# Autodesk Inventor assembly: HeadUnit
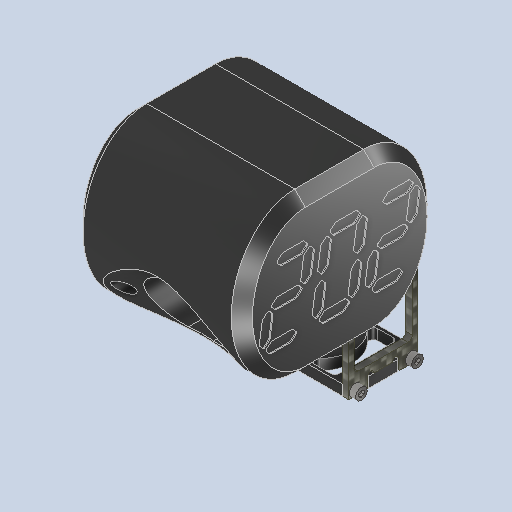
[picture p0: Inventor's stored thumbnail of the model, 512x512]
Saved by Autodesk Inventor 2024.2 (Build 282272000, 272)
## iProperties
Created: 2024-01-19
Part Number: HeadUnit
Document SubType Name: Assembly
Designer: Masato Kubotera
Mass: 257.797 g
Surface Area: 969.022 cm^2
Volume: 207.363 cm^3
Density: 1.24322 g/cm^3
Author: Masato Kubotera
## Documents named in this file (17)
- C:\Users\masato\OneDrive - Chiba Institute of Technology\CIT Brains\RoboCup2024\Mechanic\SUSTAINA-OP2-DEV - 作業\NativeFiles\Boby\Head\HeadUnit.iam
- C:\Users\masato\OneDrive - Chiba Institute of Technology\CIT Brains\RoboCup2024\Mechanic\SUSTAINA-OP2-DEV - 作業\NativeFiles\Boby\COTS\Screws\CapScrew\UC-0308.ipt
- C:\Users\masato\OneDrive - Chiba Institute of Technology\CIT Brains\RoboCup2024\Mechanic\SUSTAINA-OP2-DEV - 作業\NativeFiles\Boby\Head\HeadCameraMountFrame.ipt
- C:\Users\masato\OneDrive - Chiba Institute of Technology\CIT Brains\RoboCup2024\Mechanic\SUSTAINA-OP2-DEV - 作業\NativeFiles\Boby\Head\HeadHornFrame.ipt
- C:\Users\masato\OneDrive - Chiba Institute of Technology\CIT Brains\RoboCup2024\Mechanic\SUSTAINA-OP2-DEV - 作業\NativeFiles\Boby\Head\HeadSideFrame.ipt
- C:\Users\masato\OneDrive - Chiba Institute of Technology\CIT Brains\RoboCup2024\Mechanic\SUSTAINA-OP2-DEV - 作業\NativeFiles\Boby\COTS\Spacers\C-2006-4.ipt
- C:\Users\masato\OneDrive - Chiba Institute of Technology\CIT Brains\RoboCup2024\Mechanic\SUSTAINA-OP2-DEV - 作業\NativeFiles\Boby\Head\HeadSpeakerMountFrame.ipt
- C:\Users\masato\OneDrive - Chiba Institute of Technology\CIT Brains\RoboCup2024\Mechanic\SUSTAINA-OP2-DEV - 作業\NativeFiles\Boby\COTS\ElectronicComponents\CMS-402811-28SP.ipt
- C:\Users\masato\OneDrive - Chiba Institute of Technology\CIT Brains\RoboCup2024\Mechanic\SUSTAINA-OP2-DEV - 作業\NativeFiles\Boby\Head\HeadCircuitMountFrame.ipt
- C:\Users\masato\OneDrive - Chiba Institute of Technology\CIT Brains\RoboCup2024\Mechanic\SUSTAINA-OP2-DEV - 作業\NativeFiles\Boby\COTS\Screws\CapScrew\UC-0206.ipt
- C:\Users\masato\OneDrive - Chiba Institute of Technology\CIT Brains\RoboCup2024\Mechanic\SUSTAINA-OP2-DEV - 作業\NativeFiles\Boby\Head\HeadCover.ipt
- C:\Users\masato\OneDrive - Chiba Institute of Technology\CIT Brains\RoboCup2024\Mechanic\SUSTAINA-OP2-DEV - 作業\NativeFiles\Boby\COTS\ElectronicComponents\Cameras\e-CAM50_CUONX.ipt
- C:\Users\masato\OneDrive - Chiba Institute of Technology\CIT Brains\RoboCup2024\Mechanic\SUSTAINA-OP2-DEV - 作業\NativeFiles\Boby\COTS\Spacers\C-2002.5-4.ipt
- C:\Users\masato\OneDrive - Chiba Institute of Technology\CIT Brains\RoboCup2024\Mechanic\SUSTAINA-OP2-DEV - 作業\NativeFiles\Boby\COTS\Screws\CapScrew\FC-0215EB.ipt
- C:\Users\masato\OneDrive - Chiba Institute of Technology\CIT Brains\RoboCup2024\Mechanic\SUSTAINA-OP2-DEV - 作業\NativeFiles\Boby\CustomPCBs\SUSTAINA-SCI-TO-HDMI-BOARD.ipt
- C:\Users\masato\OneDrive - Chiba Institute of Technology\CIT Brains\RoboCup2024\Mechanic\SUSTAINA-OP2-DEV - 作業\NativeFiles\Boby\COTS\CIL926-F2.4-M12A650.ipt
- C:\Users\masato\OneDrive - Chiba Institute of Technology\CIT Brains\RoboCup2024\Mechanic\SUSTAINA-OP2-DEV - 作業\NativeFiles\Boby\COTS\Screws\CapScrew\UC-0310.ipt
## Components (50 placed, 16 different names)
1. HeadSpeakerMountFrame:1 — Insert:58, Insert:59, Insert:60, Insert:61, Insert:66, Insert:67, Insert:68, Insert:69
2. HeadCircuitMountFrame:1 — Insert:74, Insert:75, Insert:76, Insert:77, Insert:94, Insert:95
3. HeadCameraMountFrame:1 — Insert:37, Insert:38, Insert:39, Insert:40, Insert:92, Insert:93
4. HeadSideFrame:1 — Insert:29, Insert:30, Insert:31, Insert:32, Insert:37, Insert:38, Insert:42, Insert:43, Insert:58, Insert:59, Insert:62, Insert:63, Insert:74, Insert:75, Insert:82, Insert:83
5. HeadSideFrame:2 — Insert:33, Insert:34, Insert:35, Insert:36, Insert:39, Insert:40, Insert:44, Insert:45, Insert:60, Insert:61, Insert:64, Insert:65, Insert:76, Insert:77, Insert:84, Insert:85
6. HeadHornFrame:1 — Mate:1, Angle:1, Mate:2, Insert:24, Insert:25, Insert:26, Insert:29, Insert:30, Insert:33, Insert:34
7. SUSTAINA-SCI-TO-HDMI-BOARD:1 — Insert:94, Insert:95, Insert:96, Insert:97
8. HeadCover:1 — Insert:121, Insert:122
9. CMS-402811-28SP:1 — Insert:66, Insert:67, Insert:68, Insert:69, Insert:70, Insert:71, Insert:72, Insert:73
10. CIL926-F2.4-M12A650:1 — Insert:118
11. e-CAM50_CUONX:1 — Insert:108, Insert:109, Insert:110, Insert:111, Insert:112, Insert:113, Insert:114, Insert:115, Insert:116, Insert:117, Insert:118, Insert:119, Insert:120
12. FC-0215EB:1 — Insert:108
13. FC-0215EB:2 — Insert:110
14. FC-0215EB:3 — Insert:112
15. FC-0215EB:4 — Insert:114
16. UC-0308:1 — Insert:31
17. UC-0308:2 — Insert:32
18. UC-0308:3 — Insert:36
19. UC-0308:4 — Insert:35
20. UC-0308:6 — Insert:24
21. UC-0308:7 — Insert:25
22. UC-0308:8 — Insert:26
23. UC-0308:9 — Insert:70
24. UC-0308:10 — Insert:71
25. UC-0308:11 — Insert:72
26. UC-0308:12 — Insert:73
27. UC-0206:3 — Insert:42
28. UC-0206:4 — Insert:43
29. UC-0206:5 — Insert:62
30. UC-0206:6 — Insert:63
31. UC-0206:7 — Insert:44
32. UC-0206:8 — Insert:45
33. UC-0206:9 — Insert:64
34. UC-0206:10 — Insert:65
35. UC-0206:11 — Insert:82
36. UC-0206:12 — Insert:83
37. UC-0206:13 — Insert:84
38. UC-0206:14 — Insert:85
39. UC-0206:15 — Insert:96
40. UC-0206:16 — Insert:97
41. UC-0310:1 — Insert:121
42. UC-0310:2 — Insert:122
43. C-2006-4:1 — Insert:109
44. C-2006-4:2 — Insert:113
45. C-2006-4:3 — Insert:111
46. C-2006-4:4 — Insert:115
47. C-2002.5-4:1 — Insert:93, Insert:116
48. C-2002.5-4:2 — Insert:92, Insert:117
49. C-2002.5-4:3 — Insert:119
50. C-2002.5-4:4 — Insert:120
## Relationships (70: Insert 64, Flush 3, Mate 2, Angle 1)
- Mate:1: HeadHornFrame:1
- Angle:1 (0 deg): HeadHornFrame:1
- Mate:2: HeadHornFrame:1
- Insert:24: HeadHornFrame:1 ↔ UC-0308:6
- Insert:25: HeadHornFrame:1 ↔ UC-0308:7
- Insert:26: HeadHornFrame:1 ↔ UC-0308:8
- Insert:29: HeadSideFrame:1 ↔ HeadHornFrame:1
- Insert:30: HeadSideFrame:1 ↔ HeadHornFrame:1
- Insert:31: HeadSideFrame:1 ↔ UC-0308:1
- Insert:32: HeadSideFrame:1 ↔ UC-0308:2
- Insert:33: HeadSideFrame:2 ↔ HeadHornFrame:1
- Insert:34: HeadSideFrame:2 ↔ HeadHornFrame:1
- Insert:35: HeadSideFrame:2 ↔ UC-0308:4
- Insert:36: HeadSideFrame:2 ↔ UC-0308:3
- Insert:37: HeadCameraMountFrame:1 ↔ HeadSideFrame:1
- Insert:38: HeadCameraMountFrame:1 ↔ HeadSideFrame:1
- Insert:39: HeadCameraMountFrame:1 ↔ HeadSideFrame:2
- Insert:40: HeadCameraMountFrame:1 ↔ HeadSideFrame:2
- Insert:42: HeadSideFrame:1 ↔ UC-0206:3
- Insert:43: HeadSideFrame:1 ↔ UC-0206:4
- Insert:44: HeadSideFrame:2 ↔ UC-0206:7
- Insert:45: HeadSideFrame:2 ↔ UC-0206:8
- [Flush]: HeadCover:1
- [Flush]: HeadCover:1
- [Flush]: HeadCover:1
- Insert:58: HeadSpeakerMountFrame:1 ↔ HeadSideFrame:1
- Insert:59: HeadSpeakerMountFrame:1 ↔ HeadSideFrame:1
- Insert:60: HeadSpeakerMountFrame:1 ↔ HeadSideFrame:2
- Insert:61: HeadSpeakerMountFrame:1 ↔ HeadSideFrame:2
- Insert:62: HeadSideFrame:1 ↔ UC-0206:5
- Insert:63: HeadSideFrame:1 ↔ UC-0206:6
- Insert:64: HeadSideFrame:2 ↔ UC-0206:9
- Insert:65: HeadSideFrame:2 ↔ UC-0206:10
- Insert:66: HeadSpeakerMountFrame:1 ↔ CMS-402811-28SP:1
- Insert:67: HeadSpeakerMountFrame:1 ↔ CMS-402811-28SP:1
- Insert:68: HeadSpeakerMountFrame:1 ↔ CMS-402811-28SP:1
- Insert:69: HeadSpeakerMountFrame:1 ↔ CMS-402811-28SP:1
- Insert:70: CMS-402811-28SP:1 ↔ UC-0308:9
- Insert:71: CMS-402811-28SP:1 ↔ UC-0308:10
- Insert:72: CMS-402811-28SP:1 ↔ UC-0308:11
- Insert:73: CMS-402811-28SP:1 ↔ UC-0308:12
- Insert:74: HeadCircuitMountFrame:1 ↔ HeadSideFrame:1
- Insert:75: HeadCircuitMountFrame:1 ↔ HeadSideFrame:1
- Insert:76: HeadCircuitMountFrame:1 ↔ HeadSideFrame:2
- Insert:77: HeadCircuitMountFrame:1 ↔ HeadSideFrame:2
- Insert:82: HeadSideFrame:1 ↔ UC-0206:11
- Insert:83: HeadSideFrame:1 ↔ UC-0206:12
- Insert:84: HeadSideFrame:2 ↔ UC-0206:13
- Insert:85: HeadSideFrame:2 ↔ UC-0206:14
- Insert:92: HeadCameraMountFrame:1 ↔ C-2002.5-4:2
- Insert:93: HeadCameraMountFrame:1 ↔ C-2002.5-4:1
- Insert:94: HeadCircuitMountFrame:1 ↔ SUSTAINA-SCI-TO-HDMI-BOARD:1
- Insert:95: HeadCircuitMountFrame:1 ↔ SUSTAINA-SCI-TO-HDMI-BOARD:1
- Insert:96: SUSTAINA-SCI-TO-HDMI-BOARD:1 ↔ UC-0206:15
- Insert:97: SUSTAINA-SCI-TO-HDMI-BOARD:1 ↔ UC-0206:16
- Insert:108: e-CAM50_CUONX:1 ↔ FC-0215EB:1
- Insert:109: e-CAM50_CUONX:1 ↔ C-2006-4:1
- Insert:110: e-CAM50_CUONX:1 ↔ FC-0215EB:2
- Insert:111: e-CAM50_CUONX:1 ↔ C-2006-4:3
- Insert:112: e-CAM50_CUONX:1 ↔ FC-0215EB:3
- Insert:113: e-CAM50_CUONX:1 ↔ C-2006-4:2
- Insert:114: e-CAM50_CUONX:1 ↔ FC-0215EB:4
- Insert:115: e-CAM50_CUONX:1 ↔ C-2006-4:4
- Insert:116: e-CAM50_CUONX:1 ↔ C-2002.5-4:1
- Insert:117: e-CAM50_CUONX:1 ↔ C-2002.5-4:2
- Insert:118 (-8 mm): CIL926-F2.4-M12A650:1 ↔ e-CAM50_CUONX:1
- Insert:119: e-CAM50_CUONX:1 ↔ C-2002.5-4:3
- Insert:120: e-CAM50_CUONX:1 ↔ C-2002.5-4:4
- Insert:121: HeadCover:1 ↔ UC-0310:1
- Insert:122: HeadCover:1 ↔ UC-0310:2
